# Autodesk Inventor assembly: bottom idler housing(right)1
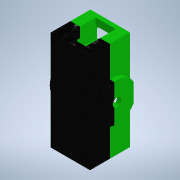
[picture p0: Inventor's stored thumbnail of the model, 180x180]
Saved by Autodesk Inventor 2020.4 (Build 244396000, 396)
## iProperties
Created: 2021-03-29
Part Number: bottom idler housing(right)1
Document SubType Name: Assembly
Designer: AOB
Mass: 32.4286 g
Surface Area: 168.027 cm^2
Volume: 30.593 cm^3
Density: 1.06 g/cm^3
Author: AOB
## Documents named in this file (3)
- C:\Users\marti\Documents\Inventor\ProjectBoron\Boron Ultima\bottom idler housing(right)1.iam
- C:\Users\marti\Documents\Inventor\ProjectBoron\Boron Ultima\bottom idler housing-A(right)1.ipt
- C:\Users\marti\Documents\Inventor\ProjectBoron\Boron Ultima\bottom idler housing-B(right)1.ipt
## Components (2 placed, 2 different names)
1. bottom idler housing-A(right)1:1 — Flush:2, Flush:1, Rigid:1
2. bottom idler housing-B(right)1:1 — Flush:2, Flush:1, Rigid:1
## Relationships (3: Flush 2, WeldJoint 1)
- Flush:2: bottom idler housing-A(right)1:1 ↔ bottom idler housing-B(right)1:1
- Flush:1: bottom idler housing-A(right)1:1 ↔ bottom idler housing-B(right)1:1
- Rigid:1 [WeldJoint]: bottom idler housing-A(right)1:1 ↔ bottom idler housing-B(right)1:1
